# Autodesk Inventor assembly: PoGo_connector
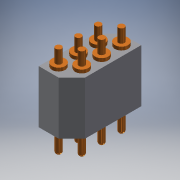
[picture p0: Inventor's stored thumbnail of the model, 180x180]
Saved by Autodesk Inventor 2019 (Build 230136000, 136)
## iProperties
Created: 2018-10-20
Part Number: PoGo_connector
Material: Generisch
Document SubType Name: Assembly
Designer: WhoTheHeck
Author: WhoTheHeck
## Documents named in this file (3)
- E:\Dokumente\PG+Ext\Modell\PoGo_Con\PoGo_connector.iam
- E:\Dokumente\PG+Ext\Modell\PoGo_Con\con_case.ipt
- E:\Dokumente\PG+Ext\Modell\PoGo_Con\PoGo_pin.ipt
## Components (7 placed, 2 different names)
1. con_case:1 — Passend:1, Passend:2, Passend:3, Passend:4, Passend:5, Passend:6, Passend:7, Passend:8, Passend:9, Passend:10, Passend:11, Passend:12
2. PoGo_pin:1 — Passend:1, Passend:7
3. PoGo_pin:2 — Passend:2, Passend:8
4. PoGo_pin:3 — Passend:3, Passend:9
5. PoGo_pin:4 — Passend:4, Passend:10
6. PoGo_pin:5 — Passend:5, Passend:11
7. PoGo_pin:6 — Passend:6, Passend:12
## Relationships (12: Mate 12)
- Passend:1 [Mate]: con_case:1 ↔ PoGo_pin:1
- Passend:2 [Mate]: con_case:1 ↔ PoGo_pin:2
- Passend:3 [Mate]: con_case:1 ↔ PoGo_pin:3
- Passend:4 [Mate]: con_case:1 ↔ PoGo_pin:4
- Passend:5 [Mate]: con_case:1 ↔ PoGo_pin:5
- Passend:6 [Mate]: con_case:1 ↔ PoGo_pin:6
- Passend:7 [Mate]: con_case:1 ↔ PoGo_pin:1
- Passend:8 [Mate]: con_case:1 ↔ PoGo_pin:2
- Passend:9 [Mate]: con_case:1 ↔ PoGo_pin:3
- Passend:10 [Mate]: con_case:1 ↔ PoGo_pin:4
- Passend:11 [Mate]: con_case:1 ↔ PoGo_pin:5
- Passend:12 [Mate]: con_case:1 ↔ PoGo_pin:6
